# Autodesk Inventor assembly: Chassis-ver12-1111-2019
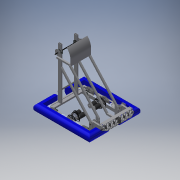
[picture p0: Inventor's stored thumbnail of the model, 180x180]
Saved by Autodesk Inventor 2018 (Build 220112000, 112)
## iProperties
Created: 2019-10-10
Part Number: Chassis-ver12-1111-2019
Document SubType Name: Assembly
Designer: JMHal
Author: JMHal
## Documents named in this file (18)
- E:\GrabCAD\Power Hawks CAD\2020 Infinite Recharge\Chassis\Assembly\Chassis-ver12-1111-2019.iam
- E:\GrabCAD\Power Hawks CAD\2020 Infinite Recharge\Chassis\Parts\2x1 20in Alluminum with Cal Drop.ver1-1111-2019.ipt
- E:\GrabCAD\Power Hawks CAD\2020 Infinite Recharge\Chassis\Parts\2x1 20in Alluminum.ver1-1111-2019.ipt
- E:\GrabCAD\Power Hawks CAD\2020 Infinite Recharge\Chassis\Parts\2x1 2in Alluminum Block.ver1-1111-2019.ipt
- E:\GrabCAD\Power Hawks CAD\Resources\VEXpro Resources\Bearings\0.5inHexFlangedBearing(1.125inx0.313in)-1111-2016.ipt
- E:\GrabCAD\Power Hawks CAD\Resources\VEXpro Resources\Versa Motion\VersaBlockKit-1111-2016.ipt
- E:\GrabCAD\Power Hawks CAD\Resources\VEXpro Resources\Gearboxes\WCP SS Gearbox\SS-Gearbox.iam
- E:\GrabCAD\Power Hawks CAD\Resources\VEXpro Resources\Gussets\ChassisGusset-1111-2016.ipt
- E:\GrabCAD\Power Hawks CAD\Resources\VEXpro Resources\Spacers\0.5inAcetalSpace(0.5inHex)-1111-2016.ipt
- E:\GrabCAD\Power Hawks CAD\Resources\VEXpro Resources\Wheels\6 inch\6x1inTractionWheel-1111-2016.iam
- E:\GrabCAD\Power Hawks CAD\2020 Infinite Recharge\Chassis\Parts\Bumbers.ver1-1111-2019.ipt
- E:\GrabCAD\Power Hawks CAD\Season Archives\2019 - Deep Space\Chassis\Parts\AluminumBracket.ipt
- E:\GrabCAD\Power Hawks CAD\2020 Infinite Recharge\Chassis\Parts\BumperMount1-ver1-1111-2019.ipt
- E:\GrabCAD\Power Hawks CAD\2020 Infinite Recharge\Intake\Assemblies\IntakeAssembly-ver1-1111-2020.iam
- E:\GrabCAD\Power Hawks CAD\2020 Infinite Recharge\Platform.ver1-1111-2020.ipt
- E:\GrabCAD\Power Hawks CAD\2020 Infinite Recharge\Powercell.ver1-1111-2020.ipt
- E:\GrabCAD\Power Hawks CAD\2020 Infinite Recharge\Shooting\Assemblies\ShooterPrototype-ver2-1111-2019.iam
- E:\GrabCAD\Power Hawks CAD\2020 Infinite Recharge\Storage\Assemblies\StorageAssembly.ver4-1111-2020.iam
## Components (55 placed, 17 different names)
1. 2x1 20in Alluminum with Cal Drop.ver1-1111-2019:1 — Mate:31, Mate:32, Insert:8, Mate:53, Angle:9, Insert:19, Angle:11, Flush:1, Mate:65, Mate:66, Flush:2, Mate:67, Flush:4, Flush:5, Mate:77, Mate:78, Flush:16, Flush:17, Mate:80, Flush:20, Flush:23, Symmetry:1, Symmetry:2, Flush:62, Mate:141, Mate:146, Angle:15, Mate:147, Mate:148, Angle:16, Mate:149, Cylindrical:65, Mate:209, Angle:23, Mate:215, Flush:66
2. 2x1 20in Alluminum.ver1-1111-2019:1 — Mate:65, Mate:66, Flush:2, Mate:68, Mate:72, Mate:81, Flush:22, Mate:82, Flush:24, Flush:62, Mate:140, Flush:63, Mate:197, Mate:198, Mate:199, Mate:200, Mate:201, Mate:212
3. 2x1 20in Alluminum with Cal Drop.ver1-1111-2019:2 — Insert:5, Angle:7, Insert:23, Angle:13, Flush:6, Flush:8, Mate:73, Flush:9, Flush:34, Flush:35, Flush:36, Flush:37, Symmetry:1, Symmetry:2, Mate:142, Mate:143, Mate:156, Mate:157, Angle:17, Mate:158, Mate:159, Angle:18, Cylindrical:64, Mate:208, Angle:22, Mate:211, Flush:64, Mate:213, Flush:65
4. 2x1 20in Alluminum.ver1-1111-2019:2 — Mate:67, Flush:4, Flush:5, Mate:69, Flush:6, Mate:71, Mate:73, Mate:79, Flush:19, Flush:21, Mate:214
5. ChassisGusset-1111-2016:1 — Mate:76, Flush:12, Flush:36
6. ChassisGusset-1111-2016:2 — Mate:75, Flush:11, Flush:35
7. ChassisGusset-1111-2016:3 — Mate:78, Flush:14, Flush:17
8. ChassisGusset-1111-2016:4 — Mate:77, Flush:15, Flush:16
9. ChassisGusset-1111-2016:5 — Mate:82, Flush:24, Flush:34
10. ChassisGusset-1111-2016:6 — Mate:81, Flush:22, Flush:23
11. ChassisGusset-1111-2016:7 — Mate:80, Flush:20, Flush:21
12. ChassisGusset-1111-2016:8 — Mate:79, Flush:19, Flush:37, Mate:216
13. 0.5inAcetalSpace(0.5inHex)-1111-2016:1 — Cylindrical:59, Mate:202, Mate:203
14. 6x1inTractionWheel-1111-2016:1 [sub-assembly] — Mate:203
15. 6x1inTractionWheel-1111-2016:5 [sub-assembly]
16. Bumbers.ver1-1111-2019:1 — Mate:139, Mate:140, Mate:210
17. VersaBlockKit-1111-2016:13 — Mate:146, Angle:15, Mate:147, Rotational:17
18. VersaBlockKit-1111-2016:14 — Mate:148, Angle:16, Mate:149, Cylindrical:45, Mate:153
19. 0.5inHexFlangedBearing(1.125inx0.313in)-1111-2016:21 — Cylindrical:45, Mate:153, Cylindrical:61, Mate:205
20. 6x1inTractionWheel-1111-2016:11 [sub-assembly] — Mate:206
21. 0.5inHexFlangedBearing(1.125inx0.313in)-1111-2016:22 — Rotational:17
22. 0.5inAcetalSpace(0.5inHex)-1111-2016:3 — Cylindrical:61, Mate:205, Mate:206
23. VersaBlockKit-1111-2016:15 — Mate:156, Mate:157, Angle:17, Mate:160, Angle:19
24. VersaBlockKit-1111-2016:16 — Mate:158, Mate:159, Angle:18, Mate:161, Mate:165, Angle:21
25. 0.5inHexFlangedBearing(1.125inx0.313in)-1111-2016:23 — Mate:160, Angle:19, Cylindrical:56, Mate:195
26. 0.5inHexFlangedBearing(1.125inx0.313in)-1111-2016:24 — Mate:161, Mate:165, Angle:21
27. 0.5inAcetalSpace(0.5inHex)-1111-2016:4 — Cylindrical:56, Mate:195, Mate:196
28. 6x1inTractionWheel-1111-2016:12 [sub-assembly] — Mate:196
29. 6x1inTractionWheel-1111-2016:13 [sub-assembly]
30. 6x1inTractionWheel-1111-2016:14 [sub-assembly]
31. AluminumBracket:1 — Mate:167, Mate:168, Mate:169
32. AluminumBracket:4 — Mate:176, Mate:177, Mate:178
33. AluminumBracket:5 — Mate:179, Mate:180, Mate:181
34. AluminumBracket:7 — Mate:185, Mate:186, Mate:187
35. BumperMount1-ver1-1111-2019:2 — Mate:197, Mate:198, Mate:199, Mate:210
36. BumperMount1-ver1-1111-2019:3 — Mate:200, Mate:201
37. SS-Gearbox:1 [sub-assembly] — Cylindrical:65, Mate:209, Angle:23
38. SS-Gearbox:2 [sub-assembly] — Cylindrical:64, Mate:208, Angle:22
39. IntakeAssembly-ver1-1111-2020:1 [sub-assembly] — Mate:211, Flush:64, Mate:212
40. Platform.ver1-1111-2020:1 — Mate:213, Flush:65, Mate:214
41. Powercell.ver1-1111-2020:1
42. ShooterPrototype-ver2-1111-2019:1 [sub-assembly] — Mate:215, Flush:66, Mate:216, Mate:217, Flush:67, Mate:218
43. StorageAssembly.ver4-1111-2020:1 [sub-assembly] — Mate:217, Flush:67, Mate:218
44. 0.5inHexFlangedBearing(1.125inx0.313in)-1111-2016:19
45. 0.5inHexFlangedBearing(1.125inx0.313in)-1111-2016:7 — Insert:5, Mate:48, Mate:49
46. 0.5inHexFlangedBearing(1.125inx0.313in)-1111-2016:17 — Insert:19
47. 0.5inHexFlangedBearing(1.125inx0.313in)-1111-2016:10 — Insert:8, Mate:52, Cylindrical:59, Mate:202
48. 2x1 2in Alluminum Block.ver1-1111-2019:5 — Mate:31, Mate:32, Mate:69, Flush:15, Mate:167, Mate:168, Mate:169
49. 2x1 2in Alluminum Block.ver1-1111-2019:6 — Flush:1, Mate:68, Flush:14, Mate:141, Mate:176, Mate:177, Mate:178
50. 2x1 2in Alluminum Block.ver1-1111-2019:7 — Mate:72, Flush:9, Mate:75, Flush:11, Mate:143, Flush:63, Mate:179, Mate:180, Mate:181
51. 2x1 2in Alluminum Block.ver1-1111-2019:8 — Flush:8, Mate:71, Mate:76, Flush:12, Mate:139, Mate:142, Mate:185, Mate:186, Mate:187
52. VersaBlockKit-1111-2016:3 — Mate:48, Mate:49, Angle:7
53. VersaBlockKit-1111-2016:6 — Mate:52, Mate:53, Angle:9
54. VersaBlockKit-1111-2016:9 — Angle:11
55. VersaBlockKit-1111-2016:11 — Insert:23, Angle:13
## Relationships (131: Mate 75, Flush 29, Angle 12, Insert 6, CylindricalJoint 6, Symmetry 2, RevoluteJoint 1)
- Mate:31: 2x1 20in Alluminum with Cal Drop.ver1-1111-2019:1 ↔ 2x1 2in Alluminum Block.ver1-1111-2019:5
- Mate:32: 2x1 20in Alluminum with Cal Drop.ver1-1111-2019:1 ↔ 2x1 2in Alluminum Block.ver1-1111-2019:5
- Insert:5: 2x1 20in Alluminum with Cal Drop.ver1-1111-2019:2 ↔ 0.5inHexFlangedBearing(1.125inx0.313in)-1111-2016:7
- Mate:48: 0.5inHexFlangedBearing(1.125inx0.313in)-1111-2016:7 ↔ VersaBlockKit-1111-2016:3
- Mate:49: 0.5inHexFlangedBearing(1.125inx0.313in)-1111-2016:7 ↔ VersaBlockKit-1111-2016:3
- Insert:8: 2x1 20in Alluminum with Cal Drop.ver1-1111-2019:1 ↔ 0.5inHexFlangedBearing(1.125inx0.313in)-1111-2016:10
- Angle:7 (0 deg): 2x1 20in Alluminum with Cal Drop.ver1-1111-2019:2 ↔ VersaBlockKit-1111-2016:3
- Mate:52: 0.5inHexFlangedBearing(1.125inx0.313in)-1111-2016:10 ↔ VersaBlockKit-1111-2016:6
- Mate:53: 2x1 20in Alluminum with Cal Drop.ver1-1111-2019:1 ↔ VersaBlockKit-1111-2016:6
- Angle:9 (0 deg): 2x1 20in Alluminum with Cal Drop.ver1-1111-2019:1 ↔ VersaBlockKit-1111-2016:6
- [Mate]: 0.5inHexFlangedBearing(1.125inx0.313in)-1111-2016:17 ↔ VersaBlockKit-1111-2016:9
- [Insert]: 0.5inHexFlangedBearing(1.125inx0.313in)-1111-2016:17 ↔ VersaBlockKit-1111-2016:9
- Insert:19: 2x1 20in Alluminum with Cal Drop.ver1-1111-2019:1 ↔ 0.5inHexFlangedBearing(1.125inx0.313in)-1111-2016:17
- Angle:11 (0 deg): 2x1 20in Alluminum with Cal Drop.ver1-1111-2019:1 ↔ VersaBlockKit-1111-2016:9
- [Mate]: 0.5inHexFlangedBearing(1.125inx0.313in)-1111-2016:19 ↔ VersaBlockKit-1111-2016:11
- [Insert]: 0.5inHexFlangedBearing(1.125inx0.313in)-1111-2016:19 ↔ VersaBlockKit-1111-2016:11
- Insert:23: 2x1 20in Alluminum with Cal Drop.ver1-1111-2019:2 ↔ VersaBlockKit-1111-2016:11
- Angle:13 (0 deg): 2x1 20in Alluminum with Cal Drop.ver1-1111-2019:2 ↔ VersaBlockKit-1111-2016:11
- Flush:1: 2x1 20in Alluminum with Cal Drop.ver1-1111-2019:1 ↔ 2x1 2in Alluminum Block.ver1-1111-2019:6
- Mate:65: 2x1 20in Alluminum with Cal Drop.ver1-1111-2019:1 ↔ 2x1 20in Alluminum.ver1-1111-2019:1
- Mate:66: 2x1 20in Alluminum with Cal Drop.ver1-1111-2019:1 ↔ 2x1 20in Alluminum.ver1-1111-2019:1
- Flush:2: 2x1 20in Alluminum with Cal Drop.ver1-1111-2019:1 ↔ 2x1 20in Alluminum.ver1-1111-2019:1
- Mate:67: 2x1 20in Alluminum with Cal Drop.ver1-1111-2019:1 ↔ 2x1 20in Alluminum.ver1-1111-2019:2
- Flush:4: 2x1 20in Alluminum with Cal Drop.ver1-1111-2019:1 ↔ 2x1 20in Alluminum.ver1-1111-2019:2
- Flush:5 (-69.85 mm): 2x1 20in Alluminum with Cal Drop.ver1-1111-2019:1 ↔ 2x1 20in Alluminum.ver1-1111-2019:2
- Mate:68 (254 mm): 2x1 20in Alluminum.ver1-1111-2019:1 ↔ 2x1 2in Alluminum Block.ver1-1111-2019:6
- Mate:69 (254 mm): 2x1 20in Alluminum.ver1-1111-2019:2 ↔ 2x1 2in Alluminum Block.ver1-1111-2019:5
- Flush:6: 2x1 20in Alluminum with Cal Drop.ver1-1111-2019:2 ↔ 2x1 20in Alluminum.ver1-1111-2019:2
- Flush:8: 2x1 20in Alluminum with Cal Drop.ver1-1111-2019:2 ↔ 2x1 2in Alluminum Block.ver1-1111-2019:8
- Mate:71 (254 mm): 2x1 20in Alluminum.ver1-1111-2019:2 ↔ 2x1 2in Alluminum Block.ver1-1111-2019:8
- Mate:72 (254 mm): 2x1 20in Alluminum.ver1-1111-2019:1 ↔ 2x1 2in Alluminum Block.ver1-1111-2019:7
- Mate:73: 2x1 20in Alluminum with Cal Drop.ver1-1111-2019:2 ↔ 2x1 20in Alluminum.ver1-1111-2019:2
- Flush:9: 2x1 20in Alluminum with Cal Drop.ver1-1111-2019:2 ↔ 2x1 2in Alluminum Block.ver1-1111-2019:7
- Mate:75: ChassisGusset-1111-2016:2 ↔ 2x1 2in Alluminum Block.ver1-1111-2019:7
- Flush:11: ChassisGusset-1111-2016:2 ↔ 2x1 2in Alluminum Block.ver1-1111-2019:7
- Mate:76: ChassisGusset-1111-2016:1 ↔ 2x1 2in Alluminum Block.ver1-1111-2019:8
- Flush:12: ChassisGusset-1111-2016:1 ↔ 2x1 2in Alluminum Block.ver1-1111-2019:8
- Mate:77: 2x1 20in Alluminum with Cal Drop.ver1-1111-2019:1 ↔ ChassisGusset-1111-2016:4
- Mate:78: 2x1 20in Alluminum with Cal Drop.ver1-1111-2019:1 ↔ ChassisGusset-1111-2016:3
- Flush:14: ChassisGusset-1111-2016:3 ↔ 2x1 2in Alluminum Block.ver1-1111-2019:6
- Flush:15: ChassisGusset-1111-2016:4 ↔ 2x1 2in Alluminum Block.ver1-1111-2019:5
- Flush:16: 2x1 20in Alluminum with Cal Drop.ver1-1111-2019:1 ↔ ChassisGusset-1111-2016:4
- Flush:17: 2x1 20in Alluminum with Cal Drop.ver1-1111-2019:1 ↔ ChassisGusset-1111-2016:3
- Mate:79: 2x1 20in Alluminum.ver1-1111-2019:2 ↔ ChassisGusset-1111-2016:8
- Flush:19: 2x1 20in Alluminum.ver1-1111-2019:2 ↔ ChassisGusset-1111-2016:8
- Mate:80: 2x1 20in Alluminum with Cal Drop.ver1-1111-2019:1 ↔ ChassisGusset-1111-2016:7
- Flush:20: 2x1 20in Alluminum with Cal Drop.ver1-1111-2019:1 ↔ ChassisGusset-1111-2016:7
- Flush:21: 2x1 20in Alluminum.ver1-1111-2019:2 ↔ ChassisGusset-1111-2016:7
- Mate:81: 2x1 20in Alluminum.ver1-1111-2019:1 ↔ ChassisGusset-1111-2016:6
- Flush:22: 2x1 20in Alluminum.ver1-1111-2019:1 ↔ ChassisGusset-1111-2016:6
- Flush:23: 2x1 20in Alluminum with Cal Drop.ver1-1111-2019:1 ↔ ChassisGusset-1111-2016:6
- Mate:82: 2x1 20in Alluminum.ver1-1111-2019:1 ↔ ChassisGusset-1111-2016:5
- Flush:24: 2x1 20in Alluminum.ver1-1111-2019:1 ↔ ChassisGusset-1111-2016:5
- Flush:34: 2x1 20in Alluminum with Cal Drop.ver1-1111-2019:2 ↔ ChassisGusset-1111-2016:5
- Flush:35: 2x1 20in Alluminum with Cal Drop.ver1-1111-2019:2 ↔ ChassisGusset-1111-2016:2
- Flush:36: 2x1 20in Alluminum with Cal Drop.ver1-1111-2019:2 ↔ ChassisGusset-1111-2016:1
- Flush:37: 2x1 20in Alluminum with Cal Drop.ver1-1111-2019:2 ↔ ChassisGusset-1111-2016:8
- Symmetry:1: 2x1 20in Alluminum with Cal Drop.ver1-1111-2019:1 ↔ 2x1 20in Alluminum with Cal Drop.ver1-1111-2019:2
- Symmetry:2: 2x1 20in Alluminum with Cal Drop.ver1-1111-2019:1 ↔ 2x1 20in Alluminum with Cal Drop.ver1-1111-2019:2
- Flush:62 (69.85 mm): 2x1 20in Alluminum with Cal Drop.ver1-1111-2019:1 ↔ 2x1 20in Alluminum.ver1-1111-2019:1
- Mate:139 (-127 mm): Bumbers.ver1-1111-2019:1 ↔ 2x1 2in Alluminum Block.ver1-1111-2019:8
- Mate:140: 2x1 20in Alluminum.ver1-1111-2019:1 ↔ Bumbers.ver1-1111-2019:1
- Mate:141: 2x1 20in Alluminum with Cal Drop.ver1-1111-2019:1 ↔ 2x1 2in Alluminum Block.ver1-1111-2019:6
- Mate:142: 2x1 20in Alluminum with Cal Drop.ver1-1111-2019:2 ↔ 2x1 2in Alluminum Block.ver1-1111-2019:8
- Mate:143: 2x1 20in Alluminum with Cal Drop.ver1-1111-2019:2 ↔ 2x1 2in Alluminum Block.ver1-1111-2019:7
- Flush:63: 2x1 20in Alluminum.ver1-1111-2019:1 ↔ 2x1 2in Alluminum Block.ver1-1111-2019:7
- Mate:146: 2x1 20in Alluminum with Cal Drop.ver1-1111-2019:1 ↔ VersaBlockKit-1111-2016:13
- Angle:15 (0 deg): 2x1 20in Alluminum with Cal Drop.ver1-1111-2019:1 ↔ VersaBlockKit-1111-2016:13
- Mate:147: 2x1 20in Alluminum with Cal Drop.ver1-1111-2019:1 ↔ VersaBlockKit-1111-2016:13
- Mate:148: 2x1 20in Alluminum with Cal Drop.ver1-1111-2019:1 ↔ VersaBlockKit-1111-2016:14
- Angle:16 (0 deg): 2x1 20in Alluminum with Cal Drop.ver1-1111-2019:1 ↔ VersaBlockKit-1111-2016:14
- Mate:149: 2x1 20in Alluminum with Cal Drop.ver1-1111-2019:1 ↔ VersaBlockKit-1111-2016:14
- Cylindrical:45: VersaBlockKit-1111-2016:14 ↔ 0.5inHexFlangedBearing(1.125inx0.313in)-1111-2016:21
- Rotational:17 [RevoluteJoint]: VersaBlockKit-1111-2016:13 ↔ 0.5inHexFlangedBearing(1.125inx0.313in)-1111-2016:22
- Mate:153: VersaBlockKit-1111-2016:14 ↔ 0.5inHexFlangedBearing(1.125inx0.313in)-1111-2016:21
- Mate:156: 2x1 20in Alluminum with Cal Drop.ver1-1111-2019:2 ↔ VersaBlockKit-1111-2016:15
- Mate:157: 2x1 20in Alluminum with Cal Drop.ver1-1111-2019:2 ↔ VersaBlockKit-1111-2016:15
- Angle:17 (0 deg): 2x1 20in Alluminum with Cal Drop.ver1-1111-2019:2 ↔ VersaBlockKit-1111-2016:15
- Mate:158: 2x1 20in Alluminum with Cal Drop.ver1-1111-2019:2 ↔ VersaBlockKit-1111-2016:16
- Mate:159: 2x1 20in Alluminum with Cal Drop.ver1-1111-2019:2 ↔ VersaBlockKit-1111-2016:16
- Angle:18 (0 deg): 2x1 20in Alluminum with Cal Drop.ver1-1111-2019:2 ↔ VersaBlockKit-1111-2016:16
- Mate:160: VersaBlockKit-1111-2016:15 ↔ 0.5inHexFlangedBearing(1.125inx0.313in)-1111-2016:23
- Mate:161: VersaBlockKit-1111-2016:16 ↔ 0.5inHexFlangedBearing(1.125inx0.313in)-1111-2016:24
- Angle:19 (0 deg): VersaBlockKit-1111-2016:15 ↔ 0.5inHexFlangedBearing(1.125inx0.313in)-1111-2016:23
- Mate:165: VersaBlockKit-1111-2016:16 ↔ 0.5inHexFlangedBearing(1.125inx0.313in)-1111-2016:24
- Angle:21 (0 deg): VersaBlockKit-1111-2016:16 ↔ 0.5inHexFlangedBearing(1.125inx0.313in)-1111-2016:24
- Mate:167: AluminumBracket:1 ↔ 2x1 2in Alluminum Block.ver1-1111-2019:5
- Mate:168: AluminumBracket:1 ↔ 2x1 2in Alluminum Block.ver1-1111-2019:5
- Mate:169: AluminumBracket:1 ↔ 2x1 2in Alluminum Block.ver1-1111-2019:5
- Mate:176: AluminumBracket:4 ↔ 2x1 2in Alluminum Block.ver1-1111-2019:6
- Mate:177: AluminumBracket:4 ↔ 2x1 2in Alluminum Block.ver1-1111-2019:6
- Mate:178 (0.127 mm): AluminumBracket:4 ↔ 2x1 2in Alluminum Block.ver1-1111-2019:6
- Mate:179: AluminumBracket:5 ↔ 2x1 2in Alluminum Block.ver1-1111-2019:7
- Mate:180: AluminumBracket:5 ↔ 2x1 2in Alluminum Block.ver1-1111-2019:7
- Mate:181 (0.0762 mm): AluminumBracket:5 ↔ 2x1 2in Alluminum Block.ver1-1111-2019:7
- Mate:185: AluminumBracket:7 ↔ 2x1 2in Alluminum Block.ver1-1111-2019:8
- Mate:186: AluminumBracket:7 ↔ 2x1 2in Alluminum Block.ver1-1111-2019:8
- Mate:187 (0.6096 mm): AluminumBracket:7 ↔ 2x1 2in Alluminum Block.ver1-1111-2019:8
- Cylindrical:56: 0.5inHexFlangedBearing(1.125inx0.313in)-1111-2016:23 ↔ 0.5inAcetalSpace(0.5inHex)-1111-2016:4
- Mate:195 (6.35 mm): 0.5inHexFlangedBearing(1.125inx0.313in)-1111-2016:23 ↔ 0.5inAcetalSpace(0.5inHex)-1111-2016:4
- Mate:196: 0.5inAcetalSpace(0.5inHex)-1111-2016:4 ↔ 6x1inTractionWheel-1111-2016:12
- Mate:197: 2x1 20in Alluminum.ver1-1111-2019:1 ↔ BumperMount1-ver1-1111-2019:2
- Mate:198: 2x1 20in Alluminum.ver1-1111-2019:1 ↔ BumperMount1-ver1-1111-2019:2
- Mate:199: 2x1 20in Alluminum.ver1-1111-2019:1 ↔ BumperMount1-ver1-1111-2019:2
- Mate:200: 2x1 20in Alluminum.ver1-1111-2019:1 ↔ BumperMount1-ver1-1111-2019:3
- Mate:201: 2x1 20in Alluminum.ver1-1111-2019:1 ↔ BumperMount1-ver1-1111-2019:3
- Cylindrical:59: 0.5inAcetalSpace(0.5inHex)-1111-2016:1 ↔ 0.5inHexFlangedBearing(1.125inx0.313in)-1111-2016:10
- Mate:202 (6.35 mm): 0.5inAcetalSpace(0.5inHex)-1111-2016:1 ↔ 0.5inHexFlangedBearing(1.125inx0.313in)-1111-2016:10
- Mate:203: 0.5inAcetalSpace(0.5inHex)-1111-2016:1 ↔ 6x1inTractionWheel-1111-2016:1
- Cylindrical:61: 0.5inHexFlangedBearing(1.125inx0.313in)-1111-2016:21 ↔ 0.5inAcetalSpace(0.5inHex)-1111-2016:3
- Mate:205 (6.35 mm): 0.5inHexFlangedBearing(1.125inx0.313in)-1111-2016:21 ↔ 0.5inAcetalSpace(0.5inHex)-1111-2016:3
- Mate:206: 6x1inTractionWheel-1111-2016:11 ↔ 0.5inAcetalSpace(0.5inHex)-1111-2016:3
- Cylindrical:64: 2x1 20in Alluminum with Cal Drop.ver1-1111-2019:2 ↔ SS-Gearbox:2
- Mate:208: 2x1 20in Alluminum with Cal Drop.ver1-1111-2019:2 ↔ SS-Gearbox:2
- Angle:22 (90 deg): 2x1 20in Alluminum with Cal Drop.ver1-1111-2019:2 ↔ SS-Gearbox:2
- Cylindrical:65: 2x1 20in Alluminum with Cal Drop.ver1-1111-2019:1 ↔ SS-Gearbox:1
- Mate:209: 2x1 20in Alluminum with Cal Drop.ver1-1111-2019:1 ↔ SS-Gearbox:1
- Angle:23 (-90 deg): 2x1 20in Alluminum with Cal Drop.ver1-1111-2019:1 ↔ SS-Gearbox:1
- Mate:210: Bumbers.ver1-1111-2019:1 ↔ BumperMount1-ver1-1111-2019:2
- Mate:211: 2x1 20in Alluminum with Cal Drop.ver1-1111-2019:2 ↔ IntakeAssembly-ver1-1111-2020:1
- Flush:64 (-8.3185 mm): 2x1 20in Alluminum with Cal Drop.ver1-1111-2019:2 ↔ IntakeAssembly-ver1-1111-2020:1
- Mate:212: 2x1 20in Alluminum.ver1-1111-2019:1 ↔ IntakeAssembly-ver1-1111-2020:1
- Mate:213 (50.8 mm): 2x1 20in Alluminum with Cal Drop.ver1-1111-2019:2 ↔ Platform.ver1-1111-2020:1
- Flush:65 (-203.2 mm): 2x1 20in Alluminum with Cal Drop.ver1-1111-2019:2 ↔ Platform.ver1-1111-2020:1
- Mate:214: 2x1 20in Alluminum.ver1-1111-2019:2 ↔ Platform.ver1-1111-2020:1
- Mate:215: 2x1 20in Alluminum with Cal Drop.ver1-1111-2019:1 ↔ ShooterPrototype-ver2-1111-2019:1
- Flush:66: 2x1 20in Alluminum with Cal Drop.ver1-1111-2019:1 ↔ ShooterPrototype-ver2-1111-2019:1
- Mate:216: ChassisGusset-1111-2016:8 ↔ ShooterPrototype-ver2-1111-2019:1
- Mate:217: ShooterPrototype-ver2-1111-2019:1 ↔ StorageAssembly.ver4-1111-2020:1
- Flush:67: ShooterPrototype-ver2-1111-2019:1 ↔ StorageAssembly.ver4-1111-2020:1
- Mate:218: ShooterPrototype-ver2-1111-2019:1 ↔ StorageAssembly.ver4-1111-2020:1
## Named parameters: d93_d89_d76 = 0 mm, d94_d90 = 0 mm, d103_d89_d76 = 0 mm, d104_d90 = 0 mm
